# Autodesk Inventor assembly: FOUR STROKE ENGINE
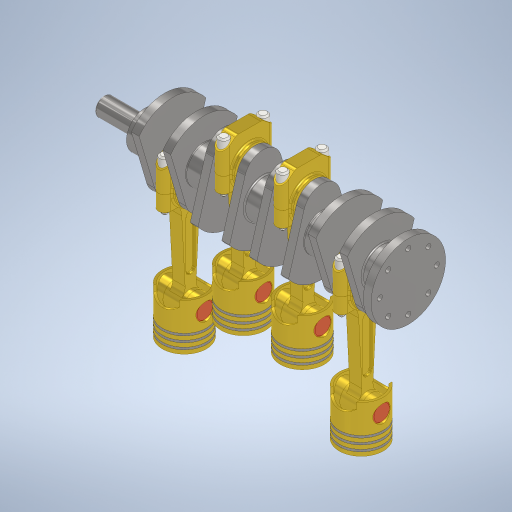
[picture p0: Inventor's stored thumbnail of the model, 512x512]
Saved by Autodesk Inventor 2023 (Build 270158000, 158)
## iProperties
Created: 2025-10-05
Part Number: FOUR STROKE ENGINE
Document SubType Name: Assembly
Designer: ayush
Author: ayush
## Documents named in this file (5)
- C:\Users\ayush\Desktop\INVENTOR FILES COLLEGE\engine\FOUR STROKE ENGINE.iam
- C:\Users\ayush\Desktop\INVENTOR FILES COLLEGE\engine\Part7 SKETCH.ipt
- C:\Users\ayush\Desktop\INVENTOR FILES COLLEGE\engine\Part2 crank shaft.ipt
- C:\Users\ayush\Desktop\INVENTOR FILES COLLEGE\engine\A.iam
- C:\Users\ayush\Desktop\INVENTOR FILES COLLEGE\engine\B.iam
## Components (10 placed, 4 different names)
1. Part7 SKETCH:1 — Mate:1, Flush:1, Mate:2, Mate:3, Mate:4, Mate:5, Mate:6
2. Part2 crank shaft:1 — Flush:1, Mate:2, Mate:7, Mate:9, Mate:10, Mate:11, Mate:12, Mate:13, Mate:14, Mate:15, Angle:1
3. A:1 [sub-assembly] — Mate:3, Mate:16
4. A:2 [sub-assembly] — Mate:4, Mate:17
5. A:3 [sub-assembly] — Mate:5, Mate:18
6. A:4 [sub-assembly] — Mate:6, Mate:19
7. B:1 [sub-assembly] — Mate:7, Mate:15, Mate:16
8. B:2 [sub-assembly] — Mate:13, Mate:14, Mate:17
9. B:3 [sub-assembly] — Mate:9, Mate:12, Mate:18
10. B:4 [sub-assembly] — Mate:10, Mate:11, Mate:19
## Relationships (20: Mate 18, Flush 1, Angle 1)
- Mate:1: Part7 SKETCH:1
- Flush:1: Part7 SKETCH:1 ↔ Part2 crank shaft:1
- Mate:2: Part7 SKETCH:1 ↔ Part2 crank shaft:1
- Mate:3: Part7 SKETCH:1 ↔ A:1
- Mate:4: Part7 SKETCH:1 ↔ A:2
- Mate:5: Part7 SKETCH:1 ↔ A:3
- Mate:6: Part7 SKETCH:1 ↔ A:4
- Mate:7: Part2 crank shaft:1 ↔ B:1
- Mate:9: Part2 crank shaft:1 ↔ B:3
- Mate:10: Part2 crank shaft:1 ↔ B:4
- Mate:11 (4 mm): Part2 crank shaft:1 ↔ B:4
- Mate:12 (4 mm): Part2 crank shaft:1 ↔ B:3
- Mate:13: Part2 crank shaft:1 ↔ B:2
- Mate:14 (4 mm): Part2 crank shaft:1 ↔ B:2
- Mate:15 (4 mm): Part2 crank shaft:1 ↔ B:1
- Mate:16: A:1 ↔ B:1
- Mate:17: A:2 ↔ B:2
- Mate:18: A:3 ↔ B:3
- Mate:19: A:4 ↔ B:4
- Angle:1 (21600 deg): Part2 crank shaft:1
